# Autodesk Inventor assembly: esp32_30pin
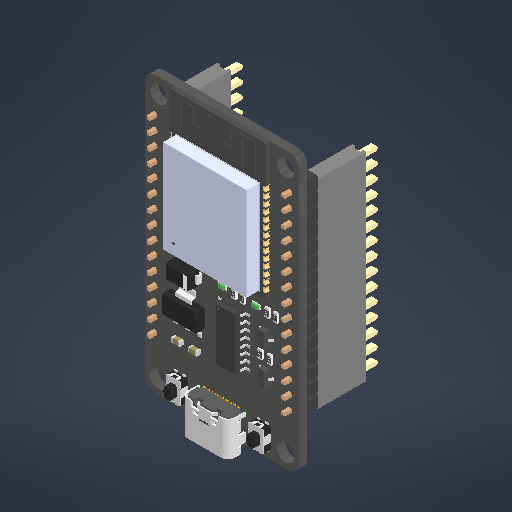
[picture p0: Inventor's stored thumbnail of the model, 512x512]
Saved by Autodesk Inventor 2026.1 (Build 301233020, 233B)
## iProperties
Created: 2023-12-08
Part Number: esp32_30pin
Document SubType Name: Assembly
Designer: celio
Sending System: Autodesk Translation Framework v12.14.0.127
Preprocessor: ST-DEVELOPER v20
Title: esp32-30pin_3dmodel_draft v1.step
## Documents named in this file (24)
- C:\Users\celio\OneDrive\Documentos\Inventor\ZeGuia\Componentes\Controlador\esp32\esp32_30pin.iam
- C:\Users\celio\OneDrive\Documentos\Inventor\ZeGuia\Componentes\Controlador\esp32\parts\Board.iam
- C:\Users\celio\OneDrive\Documentos\Inventor\ZeGuia\Componentes\Controlador\esp32\parts\Designator19.iam
- C:\Users\celio\OneDrive\Documentos\Inventor\ZeGuia\Componentes\Controlador\esp32\parts\Designator20.iam
- C:\Users\celio\OneDrive\Documentos\Inventor\ZeGuia\Componentes\Controlador\esp32\parts\Designator18.iam
- C:\Users\celio\OneDrive\Documentos\Inventor\ZeGuia\Componentes\Controlador\esp32\parts\Designator18 (1).iam
- C:\Users\celio\OneDrive\Documentos\Inventor\ZeGuia\Componentes\Controlador\esp32\parts\Designator14.iam
- C:\Users\celio\OneDrive\Documentos\Inventor\ZeGuia\Componentes\Controlador\esp32\parts\Designator9.iam
- C:\Users\celio\OneDrive\Documentos\Inventor\ZeGuia\Componentes\Controlador\esp32\parts\Designator15_1.iam
- C:\Users\celio\OneDrive\Documentos\Inventor\ZeGuia\Componentes\Controlador\esp32\parts\Designator16_1.iam
- C:\Users\celio\OneDrive\Documentos\Inventor\ZeGuia\Componentes\Controlador\esp32\parts\Designator17.iam
- C:\Users\celio\OneDrive\Documentos\Inventor\ZeGuia\Componentes\Controlador\esp32\parts\Designator16.iam
- C:\Users\celio\OneDrive\Documentos\Inventor\ZeGuia\Componentes\Controlador\esp32\parts\Designator15.iam
- C:\Users\celio\OneDrive\Documentos\Inventor\ZeGuia\Componentes\Controlador\esp32\parts\Designator14 (1).iam
- C:\Users\celio\OneDrive\Documentos\Inventor\ZeGuia\Componentes\Controlador\esp32\parts\Designator13.iam
- C:\Users\celio\OneDrive\Documentos\Inventor\ZeGuia\Componentes\Controlador\esp32\parts\Designator12.iam
- C:\Users\celio\OneDrive\Documentos\Inventor\ZeGuia\Componentes\Controlador\esp32\parts\Designator12 (1).iam
- C:\Users\celio\OneDrive\Documentos\Inventor\ZeGuia\Componentes\Controlador\esp32\parts\Designator11.iam
- C:\Users\celio\OneDrive\Documentos\Inventor\ZeGuia\Componentes\Controlador\esp32\parts\Designator10.iam
- C:\Users\celio\OneDrive\Documentos\Inventor\ZeGuia\Componentes\Controlador\esp32\parts\Designator9 (1).iam
- C:\Users\celio\OneDrive\Documentos\Inventor\ZeGuia\Componentes\Controlador\esp32\parts\Designator8.iam
- C:\Users\celio\OneDrive\Documentos\Inventor\ZeGuia\Componentes\Controlador\esp32\parts\Designator6.iam
- C:\Users\celio\OneDrive\Documentos\Inventor\ZeGuia\Componentes\Controlador\esp32\parts\Free-Models.iam
- C:\Users\celio\OneDrive\Documentos\Inventor\ZeGuia\Pinos\Femea\1x15\1x15.iam
## Components (24 placed, 23 different names)
1. Board:1 [sub-assembly]
2. Designator19:1 [sub-assembly] — Coincidente:2, Alinhado:1, Alinhado:2
3. Designator20:1 [sub-assembly] — Coincidente:1, Alinhado:3, Alinhado:4
4. Designator18:1 [sub-assembly]
5. Designator18 (1):1 [sub-assembly]
6. Designator14:1 [sub-assembly]
7. Designator9:1 [sub-assembly]
8. Designator15_1:1 [sub-assembly]
9. Designator16_1:1 [sub-assembly]
10. Designator17:1 [sub-assembly]
11. Designator16:1 [sub-assembly]
12. Designator15:1 [sub-assembly]
13. Designator14 (1):1 [sub-assembly]
14. Designator13:1 [sub-assembly]
15. Designator12:1 [sub-assembly]
16. Designator12 (1):1 [sub-assembly]
17. Designator11:1 [sub-assembly]
18. Designator10:1 [sub-assembly]
19. Designator9 (1):1 [sub-assembly]
20. Designator8:1 [sub-assembly]
21. Designator6:1 [sub-assembly]
22. Free-Models:1 [sub-assembly]
23. 1x15:1 [sub-assembly] — Coincidente:1, Alinhado:3, Alinhado:4
24. 1x15:2 [sub-assembly] — Coincidente:2, Alinhado:1, Alinhado:2
## Relationships (6: Flush 4, Mate 2)
- Coincidente:1 [Mate]: Designator20:1 ↔ 1x15:1
- Coincidente:2 [Mate]: Designator19:1 ↔ 1x15:2
- Alinhado:1 [Flush]: Designator19:1 ↔ 1x15:2
- Alinhado:2 [Flush]: Designator19:1 ↔ 1x15:2
- Alinhado:3 [Flush]: Designator20:1 ↔ 1x15:1
- Alinhado:4 [Flush]: Designator20:1 ↔ 1x15:1
